# Autodesk Inventor assembly: T01574_ASSY
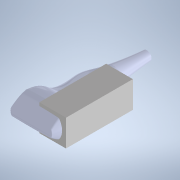
[picture p0: Inventor's stored thumbnail of the model, 180x180]
Saved by Autodesk Inventor 2022 (Build 260153000, 153)
## iProperties
Created: 2015-01-28
Part Number: T01574_ASSY
Description: STEP AP214
Document SubType Name: Assembly
Designer: biom
Sending System: SolidWorks 2014
Preprocessor: SwSTEP 2.0
Title: T01574_ASSY.STEP
Revision Number: ANY
## Documents named in this file (5)
- C:\Users\biom\Desktop\Sri\3D model\L15-7L40H-A5\T01574_ASSY.iam
- C:\Users\biom\Desktop\Sri\3D model\L15-7L40H-A5\1.ipt
- C:\Users\biom\Desktop\Sri\3D model\L15-7L40H-A5\2.ipt
- C:\Users\biom\Desktop\Sri\3D model\L15-7L40H-A5\3.ipt
- C:\Users\biom\Desktop\Sri\3D model\L15-7L40H-A5\cas1.ipt
## Components (4 placed, 4 different names)
1. 1_1
2. 2_2
3. 3_3
4. cas1:1 — Mate:1, Mate:2, Rotation/Translation:1
## Relationships (3: Mate 2, RelateRotateTranslate 1)
- Mate:1 (-15 mm): cas1:1
- Mate:2: cas1:1
- Rotation/Translation:1 [RelateRotateTranslate] (1 mm): cas1:1
